# Autodesk Inventor assembly: Frame
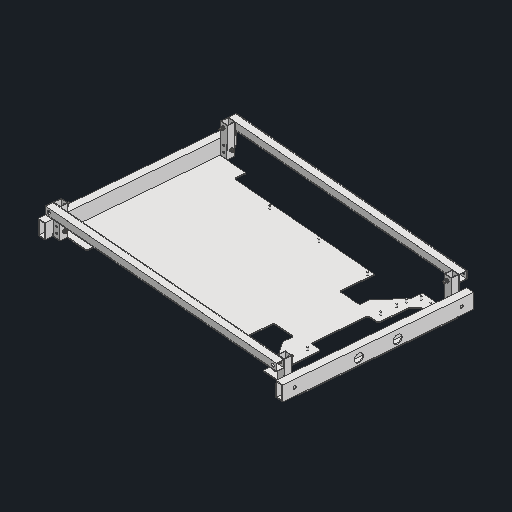
[picture p0: Inventor's stored thumbnail of the model, 512x512]
Saved by Autodesk Inventor 2022 (Build 260153000, 153)
## iProperties
Created: 2022-09-10
Part Number: Frame
Document SubType Name: Assembly
Designer: robpl
Author: robpl
## Documents named in this file (9)
- C:\Users\robpl\OneDrive\Documents\Inventor\WASP\Best Coast Drive\Frame.iam
- C:\Users\robpl\OneDrive\Documents\Inventor\WASP\Best Coast Drive\Front Bar.ipt
- C:\Users\robpl\OneDrive\Documents\Inventor\WASP\Best Coast Drive\M5 x 12.7 Rivet.ipt
- C:\Users\robpl\OneDrive\Documents\Inventor\WASP\Best Coast Drive\Back Bar.ipt
- C:\Users\robpl\OneDrive\Documents\Inventor\WASP\Best Coast Drive\Side Bar Mount.ipt
- C:\Users\robpl\OneDrive\Documents\Inventor\WASP\Best Coast Drive\Side Bar.ipt
- C:\Users\robpl\OneDrive\Documents\Inventor\Content Center Files\R2022\en-US\ISO 4762(2)\ISO 4762 - M6 x 40ISO.ipt
- C:\Users\robpl\OneDrive\Documents\Inventor\Content Center Files\R2022\en-US\ISO 7041\ISO 7041 - M6 - ISO.ipt
- C:\Users\robpl\OneDrive\Documents\Inventor\WASP\Wasp\Wasp BellyPan.ipt
## Components (51 placed, 8 different names)
1. Front Bar:1 — Mate:22, Mate:23, Mate:25, Mate:26, Mate:49, Mate:50, Mate:51, Mate:52, Mate:53, Mate:55, Mate:65, Mate:66, Mate:67, Flush:2
2. Back Bar:1 — Mate:15, Mate:16, Mate:21, Mate:24, Mate:33, Mate:34, Mate:35, Mate:36, Mate:37, Mate:39, Mate:72, Mate:73, Flush:1
3. Side Bar Mount:1 — Mate:21, Mate:24, Mate:29, Mate:38, Mate:40, Mate:46, Mate:48, Flush:1
4. Side Bar Mount:2 — Mate:15, Mate:16, Mate:30, Mate:31
5. Side Bar Mount:3 — Mate:23, Mate:25, Mate:27, Mate:28, Mate:54, Mate:56
6. Side Bar Mount:4 — Mate:22, Mate:26, Mate:32, Mate:62, Mate:64, Flush:2
7. Side Bar:1 — Mate:27, Mate:28, Mate:29, Mate:41, Mate:42, Mate:43, Mate:44, Mate:45, Mate:47
8. Side Bar:2 — Mate:30, Mate:31, Mate:32, Mate:57, Mate:58, Mate:59, Mate:60, Mate:61, Mate:63
9. Wasp BellyPan:1 — Mate:65, Mate:66, Mate:67, Mate:68, Mate:69, Mate:70, Mate:71, Mate:72, Mate:73, Mate:74, Mate:75, Mate:76, Mate:77, Mate:78, Mate:79, Mate:80, Mate:81, Mate:82, Mate:83
10. M5 x 12.7 Rivet:21 — Mate:76, Mate:77
11. M5 x 12.7 Rivet:22 — Flush:3, Mate:81
12. M5 x 12.7 Rivet:23 — Flush:3, Flush:5, Flush:6, Mate:78, Mate:79
13. M5 x 12.7 Rivet:24 — Flush:4, Mate:80
14. M5 x 12.7 Rivet:25 — Flush:6, Mate:82
15. M5 x 12.7 Rivet:26 — Flush:4, Flush:5, Mate:83
16. ISO 4762 M6 x 40:1 — Mate:33, Mate:34
17. ISO 7041 M6:1 — Mate:37, Mate:38
18. ISO 4762 M6 x 40:2 — Mate:35, Mate:36
19. ISO 7041 M6:2 — Mate:39, Mate:40
20. ISO 4762 M6 x 40:3 — Mate:41, Mate:42
21. ISO 7041 M6:3 — Mate:45, Mate:46
22. ISO 4762 M6 x 40:4 — Mate:43, Mate:44
23. ISO 7041 M6:4 — Mate:47, Mate:48
24. ISO 4762 M6 x 40:5 — Mate:49, Mate:50
25. ISO 7041 M6:5 — Mate:53, Mate:54
26. ISO 4762 M6 x 40:6 — Mate:51, Mate:52
27. ISO 7041 M6:6 — Mate:55, Mate:56
28. ISO 4762 M6 x 40:7 — Mate:57, Mate:58
29. ISO 7041 M6:7 — Mate:61, Mate:62
30. ISO 4762 M6 x 40:8 — Mate:59, Mate:60
31. ISO 7041 M6:8 — Mate:63, Mate:64
32. M5 x 12.7 Rivet:17 — Mate:74, Mate:75
33. M5 x 12.7 Rivet:18
34. M5 x 12.7 Rivet:19
35. M5 x 12.7 Rivet:20
36. M5 x 12.7 Rivet:11 — Mate:70, Mate:71
37. M5 x 12.7 Rivet:12
38. M5 x 12.7 Rivet:13
39. M5 x 12.7 Rivet:14
40. M5 x 12.7 Rivet:15
41. M5 x 12.7 Rivet:16
42. M5 x 12.7 Rivet:1 — Mate:68, Mate:69
43. M5 x 12.7 Rivet:2
44. M5 x 12.7 Rivet:3
45. M5 x 12.7 Rivet:4
46. M5 x 12.7 Rivet:5
47. M5 x 12.7 Rivet:6
48. M5 x 12.7 Rivet:7
49. M5 x 12.7 Rivet:8
50. M5 x 12.7 Rivet:9
51. M5 x 12.7 Rivet:10
## Component patterns: (4 elements, first: M5 x 12.7 Rivet:17), (6 elements, first: M5 x 12.7 Rivet:11), (10 elements, first: M5 x 12.7 Rivet:1)
## Relationships (71: Mate 65, Flush 6)
- Mate:15: Back Bar:1 ↔ Side Bar Mount:2
- Mate:16: Back Bar:1 ↔ Side Bar Mount:2
- Mate:21: Back Bar:1 ↔ Side Bar Mount:1
- Mate:22: Front Bar:1 ↔ Side Bar Mount:4
- Mate:23: Front Bar:1 ↔ Side Bar Mount:3
- Mate:24: Back Bar:1 ↔ Side Bar Mount:1
- Mate:25: Front Bar:1 ↔ Side Bar Mount:3
- Mate:26: Front Bar:1 ↔ Side Bar Mount:4
- Mate:27: Side Bar Mount:3 ↔ Side Bar:1
- Mate:28: Side Bar Mount:3 ↔ Side Bar:1
- Mate:29: Side Bar Mount:1 ↔ Side Bar:1
- Mate:30: Side Bar Mount:2 ↔ Side Bar:2
- Mate:31: Side Bar Mount:2 ↔ Side Bar:2
- Mate:32: Side Bar Mount:4 ↔ Side Bar:2
- Mate:33: Back Bar:1 ↔ ISO 4762 M6 x 40:1
- Mate:34: Back Bar:1 ↔ ISO 4762 M6 x 40:1
- Mate:35: Back Bar:1 ↔ ISO 4762 M6 x 40:2
- Mate:36: Back Bar:1 ↔ ISO 4762 M6 x 40:2
- Mate:37: Back Bar:1 ↔ ISO 7041 M6:1
- Mate:38: Side Bar Mount:1 ↔ ISO 7041 M6:1
- Mate:39: Back Bar:1 ↔ ISO 7041 M6:2
- Mate:40: Side Bar Mount:1 ↔ ISO 7041 M6:2
- Mate:41: Side Bar:1 ↔ ISO 4762 M6 x 40:3
- Mate:42: Side Bar:1 ↔ ISO 4762 M6 x 40:3
- Mate:43: Side Bar:1 ↔ ISO 4762 M6 x 40:4
- Mate:44: Side Bar:1 ↔ ISO 4762 M6 x 40:4
- Mate:45: Side Bar:1 ↔ ISO 7041 M6:3
- Mate:46: Side Bar Mount:1 ↔ ISO 7041 M6:3
- Mate:47: Side Bar:1 ↔ ISO 7041 M6:4
- Mate:48: Side Bar Mount:1 ↔ ISO 7041 M6:4
- Mate:49: Front Bar:1 ↔ ISO 4762 M6 x 40:5
- Mate:50: Front Bar:1 ↔ ISO 4762 M6 x 40:5
- Mate:51: Front Bar:1 ↔ ISO 4762 M6 x 40:6
- Mate:52: Front Bar:1 ↔ ISO 4762 M6 x 40:6
- Mate:53: Front Bar:1 ↔ ISO 7041 M6:5
- Mate:54: Side Bar Mount:3 ↔ ISO 7041 M6:5
- Mate:55: Front Bar:1 ↔ ISO 7041 M6:6
- Mate:56: Side Bar Mount:3 ↔ ISO 7041 M6:6
- Mate:57: Side Bar:2 ↔ ISO 4762 M6 x 40:7
- Mate:58: Side Bar:2 ↔ ISO 4762 M6 x 40:7
- Mate:59: Side Bar:2 ↔ ISO 4762 M6 x 40:8
- Mate:60: Side Bar:2 ↔ ISO 4762 M6 x 40:8
- Mate:61: Side Bar:2 ↔ ISO 7041 M6:7
- Mate:62: Side Bar Mount:4 ↔ ISO 7041 M6:7
- Mate:63: Side Bar:2 ↔ ISO 7041 M6:8
- Mate:64: Side Bar Mount:4 ↔ ISO 7041 M6:8
- Mate:65: Front Bar:1 ↔ Wasp BellyPan:1
- Mate:66: Front Bar:1 ↔ Wasp BellyPan:1
- Mate:67: Front Bar:1 ↔ Wasp BellyPan:1
- Mate:68: Wasp BellyPan:1 ↔ M5 x 12.7 Rivet:1
- Mate:69: Wasp BellyPan:1 ↔ M5 x 12.7 Rivet:1
- Mate:70: Wasp BellyPan:1 ↔ M5 x 12.7 Rivet:11
- Mate:71: Wasp BellyPan:1 ↔ M5 x 12.7 Rivet:11
- Mate:72: Back Bar:1 ↔ Wasp BellyPan:1
- Mate:73: Back Bar:1 ↔ Wasp BellyPan:1
- Flush:1: Back Bar:1 ↔ Side Bar Mount:1
- Flush:2: Front Bar:1 ↔ Side Bar Mount:4
- Mate:74: Wasp BellyPan:1 ↔ M5 x 12.7 Rivet:17
- Mate:75: Wasp BellyPan:1 ↔ M5 x 12.7 Rivet:17
- Mate:76: Wasp BellyPan:1 ↔ M5 x 12.7 Rivet:21
- Mate:77: Wasp BellyPan:1 ↔ M5 x 12.7 Rivet:21
- Flush:3: M5 x 12.7 Rivet:22 ↔ M5 x 12.7 Rivet:23
- Flush:4: M5 x 12.7 Rivet:24 ↔ M5 x 12.7 Rivet:26
- Flush:5: M5 x 12.7 Rivet:23 ↔ M5 x 12.7 Rivet:26
- Flush:6: M5 x 12.7 Rivet:23 ↔ M5 x 12.7 Rivet:25
- Mate:78: Wasp BellyPan:1 ↔ M5 x 12.7 Rivet:23
- Mate:79: Wasp BellyPan:1 ↔ M5 x 12.7 Rivet:23
- Mate:80: Wasp BellyPan:1 ↔ M5 x 12.7 Rivet:24
- Mate:81: Wasp BellyPan:1 ↔ M5 x 12.7 Rivet:22
- Mate:82: Wasp BellyPan:1 ↔ M5 x 12.7 Rivet:25
- Mate:83: Wasp BellyPan:1 ↔ M5 x 12.7 Rivet:26
